# Autodesk Inventor assembly: SUBChainTensioner
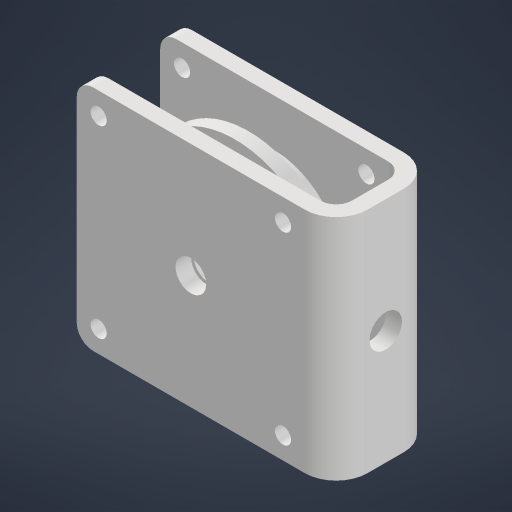
[picture p0: Inventor's stored thumbnail of the model, 512x512]
Saved by Autodesk Inventor 2024 (Build 280153000, 153)
## iProperties
Created: 2025-02-08
Part Number: SUBChainTensioner
Document SubType Name: Assembly
Designer: Tommy Rohmann
Author: Tommy Rohmann
## Documents named in this file (3)
- C:\Users\Tommy Rohmann\OneDrive\Projects\Microgravity-Press-Washing-Machine\System Design and Documentation\Inventor Design Project\SUBChainTensioner.iam
- C:\Users\Tommy Rohmann\OneDrive\Projects\Microgravity-Press-Washing-Machine\System Design and Documentation\Inventor Design Project\TensionerSprocket.ipt
- C:\Users\Tommy Rohmann\OneDrive\Projects\Microgravity-Press-Washing-Machine\System Design and Documentation\Inventor Design Project\TensionerBracket.ipt
## Components (2 placed, 2 different names)
1. TensionerSprocket:1 — Mate:1, Mate:2
2. TensionerBracket:1 — Mate:1, Mate:2
## Relationships (2: Mate 2)
- Mate:1: TensionerSprocket:1 ↔ TensionerBracket:1
- Mate:2: TensionerSprocket:1 ↔ TensionerBracket:1
